# Autodesk Inventor assembly: カート
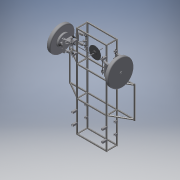
[picture p0: Inventor's stored thumbnail of the model, 180x180]
Saved by Autodesk Inventor 2018 (Build 220112000, 112)
## iProperties
Created: 2017-10-07
Part Number: カート
Material: 一般
Document SubType Name: Assembly
Designer: Kosei
Author: Kosei
## Documents named in this file (14)
- D:\Works\RBBR\CAD\カート.iam
- D:\Works\RBBR\CAD\シャーシ\シャーシ.iam
- D:\Works\RBBR\CAD\サスペンション\上アーム(前).iam
- D:\Works\RBBR\CAD\汎用部品\シャフト12x300mm.ipt
- D:\Works\RBBR\CAD\サスペンション\下アーム(前後).iam
- D:\Works\RBBR\CAD\サスペンション\車軸受け(前,左).iam
- D:\Works\RBBR\CAD\汎用部品\シャフト10x230mm.ipt
- D:\Works\RBBR\CAD\サスペンション\スプリング\スプリング.iam
- D:\Works\RBBR\CAD\車輪\前輪.ipt
- D:\Works\RBBR\CAD\車輪\前輪シャフト.ipt
- D:\Works\RBBR\CAD\車輪\前輪シャフトワッシャー.ipt
- D:\Works\RBBR\CAD\サスペンション\車軸受け(前,右).iam
- D:\Works\RBBR\CAD\ステアリング\ロッド.iam
- D:\Works\RBBR\CAD\ステアリング\車輪側スプロケット.ipt
## Components (25 placed, 13 different names)
1. シャーシ:1 [sub-assembly] — フラッシュ:2, フラッシュ:3, フラッシュ:4, 円柱状:1, フラッシュ:5, 円柱状:2, フラッシュ:6, 円柱状:3, フラッシュ:7, 円柱状:4, フラッシュ:8, メイト:1, メイト:2, メイト:3, メイト:4, フラッシュ:9, フラッシュ:10, メイト:5, フラッシュ:11, メイト:6, フラッシュ:12, 角度:3
2. シャフト12x300mm:1 — 円柱状:1, フラッシュ:5, 円柱状:5, 円柱状:11
3. シャフト12x300mm:3 — 円柱状:3, フラッシュ:7, 円柱状:7
4. シャフト10x230mm:1 — 円柱状:9, フラッシュ:9, 円柱状:12
5. 上アーム(前):1 [sub-assembly] — 円柱状:5, メイト:1, リジッド:1
6. 下アーム(前後):1 [sub-assembly] — 円柱状:7, メイト:3, リジッド:2, 円柱状:9
7. 車軸受け(前,左):1 [sub-assembly] — リジッド:1, リジッド:2, 回転:2, リジッド:9
8. スプリング:1 [sub-assembly] — 円柱状:11, 円柱状:12
9. 前輪:1 — 回転:1, リジッド:5
10. 前輪シャフト:1 — 回転:1
11. 前輪シャフトワッシャー:1 — リジッド:5, 回転:2
12. シャフト12x300mm:2 — 円柱状:2, フラッシュ:6, 円柱状:6, 円柱状:13
13. シャフト12x300mm:4 — 円柱状:4, フラッシュ:8, 円柱状:8
14. シャフト10x230mm:2 — フラッシュ:10, 円柱状:10, 円柱状:14
15. 上アーム(前):2 [sub-assembly] — 円柱状:6, メイト:2, リジッド:3
16. 下アーム(前後):2 [sub-assembly] — 円柱状:8, メイト:4, リジッド:4, 円柱状:10
17. 車軸受け(前,右):1 [sub-assembly] — リジッド:3, リジッド:4, 回転:3, リジッド:8
18. スプリング:2 [sub-assembly] — 円柱状:13, 円柱状:14
19. 前輪:2 — リジッド:6, リジッド:7
20. 前輪シャフト:2 — リジッド:6
21. 前輪シャフトワッシャー:2 — リジッド:7, 回転:3
22. ロッド:1 [sub-assembly] — リジッド:8, リジッド:12, 角度:1
23. ロッド:2 [sub-assembly] — リジッド:9, リジッド:13, 角度:2
24. 車輪側スプロケット:1 — 円柱状:15, フラッシュ:12, リジッド:12, リジッド:13, 角度:1, 角度:2, 角度:3
25. シャフト12x300mm:5 — メイト:5, フラッシュ:11, メイト:6, 円柱状:15
## Relationships (49: CylindricalJoint 15, Flush 11, WeldJoint 11, Mate 6, RevoluteJoint 3, Angle 3)
- フラッシュ:2 [Flush]: シャーシ:1
- フラッシュ:3 [Flush]: シャーシ:1
- フラッシュ:4 [Flush]: シャーシ:1
- 円柱状:1 [CylindricalJoint]: シャーシ:1 ↔ シャフト12x300mm:1
- フラッシュ:5 [Flush]: シャーシ:1 ↔ シャフト12x300mm:1
- 円柱状:2 [CylindricalJoint]: シャーシ:1 ↔ シャフト12x300mm:2
- フラッシュ:6 [Flush]: シャーシ:1 ↔ シャフト12x300mm:2
- 円柱状:3 [CylindricalJoint]: シャーシ:1 ↔ シャフト12x300mm:3
- フラッシュ:7 [Flush]: シャーシ:1 ↔ シャフト12x300mm:3
- 円柱状:4 [CylindricalJoint]: シャーシ:1 ↔ シャフト12x300mm:4
- フラッシュ:8 [Flush]: シャーシ:1 ↔ シャフト12x300mm:4
- 円柱状:5 [CylindricalJoint]: シャフト12x300mm:1 ↔ 上アーム(前):1
- メイト:1 [Mate]: シャーシ:1 ↔ 上アーム(前):1
- 円柱状:6 [CylindricalJoint]: シャフト12x300mm:2 ↔ 上アーム(前):2
- メイト:2 [Mate]: シャーシ:1 ↔ 上アーム(前):2
- 円柱状:7 [CylindricalJoint]: シャフト12x300mm:3 ↔ 下アーム(前後):1
- メイト:3 [Mate]: シャーシ:1 ↔ 下アーム(前後):1
- 円柱状:8 [CylindricalJoint]: シャフト12x300mm:4 ↔ 下アーム(前後):2
- メイト:4 [Mate]: シャーシ:1 ↔ 下アーム(前後):2
- リジッド:1 [WeldJoint]: 上アーム(前):1 ↔ 車軸受け(前,左):1
- リジッド:2 [WeldJoint]: 下アーム(前後):1 ↔ 車軸受け(前,左):1
- リジッド:3 [WeldJoint]: 上アーム(前):2 ↔ 車軸受け(前,右):1
- リジッド:4 [WeldJoint]: 下アーム(前後):2 ↔ 車軸受け(前,右):1
- 円柱状:9 [CylindricalJoint]: シャフト10x230mm:1 ↔ 下アーム(前後):1
- フラッシュ:9 [Flush]: シャーシ:1 ↔ シャフト10x230mm:1
- フラッシュ:10 [Flush]: シャーシ:1 ↔ シャフト10x230mm:2
- 円柱状:10 [CylindricalJoint]: シャフト10x230mm:2 ↔ 下アーム(前後):2
- 円柱状:11 [CylindricalJoint]: シャフト12x300mm:1 ↔ スプリング:1
- 円柱状:12 [CylindricalJoint]: シャフト10x230mm:1 ↔ スプリング:1
- 円柱状:13 [CylindricalJoint]: シャフト12x300mm:2 ↔ スプリング:2
- 円柱状:14 [CylindricalJoint]: シャフト10x230mm:2 ↔ スプリング:2
- 回転:1 [RevoluteJoint]: 前輪:1 ↔ 前輪シャフト:1
- リジッド:5 [WeldJoint]: 前輪:1 ↔ 前輪シャフトワッシャー:1
- 回転:2 [RevoluteJoint]: 車軸受け(前,左):1 ↔ 前輪シャフトワッシャー:1
- リジッド:6 [WeldJoint]: 前輪:2 ↔ 前輪シャフト:2
- リジッド:7 [WeldJoint]: 前輪:2 ↔ 前輪シャフトワッシャー:2
- 回転:3 [RevoluteJoint]: 車軸受け(前,右):1 ↔ 前輪シャフトワッシャー:2
- リジッド:8 [WeldJoint]: 車軸受け(前,右):1 ↔ ロッド:1
- リジッド:9 [WeldJoint]: 車軸受け(前,左):1 ↔ ロッド:2
- メイト:5 [Mate]: シャーシ:1 ↔ シャフト12x300mm:5
- フラッシュ:11 [Flush]: シャーシ:1 ↔ シャフト12x300mm:5
- メイト:6 [Mate]: シャーシ:1 ↔ シャフト12x300mm:5
- 円柱状:15 [CylindricalJoint]: 車輪側スプロケット:1 ↔ シャフト12x300mm:5
- フラッシュ:12 [Flush] (150 mm): シャーシ:1 ↔ 車輪側スプロケット:1
- リジッド:12 [WeldJoint]: ロッド:1 ↔ 車輪側スプロケット:1
- リジッド:13 [WeldJoint]: ロッド:2 ↔ 車輪側スプロケット:1
- 角度:1 [Angle] (0 deg): ロッド:1 ↔ 車輪側スプロケット:1
- 角度:2 [Angle] (0 deg): ロッド:2 ↔ 車輪側スプロケット:1
- 角度:3 [Angle] (0 deg): シャーシ:1 ↔ 車輪側スプロケット:1
